# Autodesk Inventor assembly: Base Cover Assembly
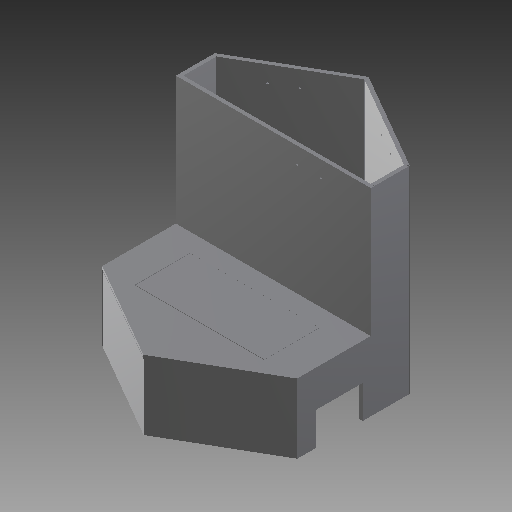
[picture p0: Inventor's stored thumbnail of the model, 512x512]
Saved by Autodesk Inventor 2017 (Build 210142000, 142)
## iProperties
Created: 2018-10-18
Part Number: Base Cover Assembly
Document SubType Name: Assembly
Designer: Dell
Author: Dell
## Documents named in this file (13)
- C:\Users\Dell\Documents\GitHub\tr2\Base\Base Cover Assembly.iam
- C:\Users\Dell\Documents\GitHub\tr2\Base\BA03.ipt
- C:\Users\Dell\Documents\GitHub\tr2\Base\BA04.ipt
- C:\Users\Dell\Documents\GitHub\tr2\Base\BA05.ipt
- C:\Users\Dell\Documents\GitHub\tr2\Base\BA10.ipt
- C:\Users\Dell\Documents\GitHub\tr2\Base\BA14.ipt
- C:\Users\Dell\Documents\GitHub\tr2\Base\Power Switch\Power Switch.iam
- C:\Users\Dell\Documents\GitHub\tr2\Base\Ethernet Port.ipt
- C:\Users\Dell\Documents\GitHub\tr2\Base\HDMI Port.ipt
- C:\Users\Dell\Documents\GitHub\tr2\Base\USB Hub.ipt
- C:\Users\Dell\Documents\GitHub\tr2\Base\BA19.ipt
- C:\Users\Dell\Documents\GitHub\tr2\Base\BA25.ipt
- C:\Users\Dell\Documents\GitHub\tr2\Base\BA26.ipt
## Components (13 placed, 12 different names)
1. BA04:1 — Flush:19, Mate:78, Mate:80, Mate:92, Flush:22
2. BA05:1 — Mate:74, Flush:18, Mate:77, Mate:82, Mate:91, Flush:20, Flush:21
3. BA03:5 — Mate:47, Flush:15, Mate:74, Mate:75
4. BA10:1 — Flush:18, Mate:77, Mate:81, Mate:83, Mate:84, Mate:87, Mate:89, Mate:90, Mate:93
5. BA14:1 — Mate:47, Mate:57, Mate:58, Mate:59, Mate:67, Mate:68, Flush:11, Mate:69, Mate:70, Mate:71, Mate:72, Flush:12, Flush:13, Flush:15, Mate:75, Flush:19, Mate:78, Mate:86
6. Power Switch:1 [sub-assembly] — Mate:57, Mate:58, Mate:59
7. Ethernet Port:1 — Mate:69, Mate:72, Flush:13
8. HDMI Port:1 — Mate:70, Mate:71, Flush:12
9. USB Hub:1 — Mate:67, Mate:68, Flush:11
10. BA19:2 — Mate:91, Flush:20, Flush:21, Mate:92, Mate:93, Flush:22
11. BA25:1 — Mate:80, Mate:81, Mate:88
12. BA25:2 — Mate:82, Mate:83, Mate:85, Mate:88
13. BA26:1 — Mate:89, Mate:90
## Relationships (37: Mate 28, Flush 9)
- Mate:47: BA03:5 ↔ BA14:1
- Mate:57: BA14:1 ↔ Power Switch:1
- Mate:58: BA14:1 ↔ Power Switch:1
- Mate:59: BA14:1 ↔ Power Switch:1
- Mate:67: BA14:1 ↔ USB Hub:1
- Mate:68: BA14:1 ↔ USB Hub:1
- Flush:11 (1 mm): BA14:1 ↔ USB Hub:1
- Mate:69: BA14:1 ↔ Ethernet Port:1
- Mate:70 (1 mm): BA14:1 ↔ HDMI Port:1
- Mate:71 (1 mm): BA14:1 ↔ HDMI Port:1
- Mate:72: BA14:1 ↔ Ethernet Port:1
- Flush:12: BA14:1 ↔ HDMI Port:1
- Flush:13: BA14:1 ↔ Ethernet Port:1
- Flush:15: BA03:5 ↔ BA14:1
- Mate:74: BA05:1 ↔ BA03:5
- Mate:75: BA03:5 ↔ BA14:1
- Flush:18: BA05:1 ↔ BA10:1
- Mate:77: BA05:1 ↔ BA10:1
- Flush:19: BA04:1 ↔ BA14:1
- Mate:78: BA04:1 ↔ BA14:1
- Mate:80: BA04:1 ↔ BA25:1
- Mate:81: BA10:1 ↔ BA25:1
- Mate:82: BA05:1 ↔ BA25:2
- Mate:83: BA10:1 ↔ BA25:2
- Mate:84: BA10:1
- Mate:85: BA25:2
- Mate:86: BA14:1
- Mate:87: BA10:1
- Mate:88: BA25:1 ↔ BA25:2
- Mate:89: BA10:1 ↔ BA26:1
- Mate:90 (1 mm): BA10:1 ↔ BA26:1
- Mate:91: BA05:1 ↔ BA19:2
- Flush:20: BA05:1 ↔ BA19:2
- Flush:21: BA05:1 ↔ BA19:2
- Mate:92: BA04:1 ↔ BA19:2
- Mate:93: BA10:1 ↔ BA19:2
- Flush:22: BA04:1 ↔ BA19:2
